# Autodesk Inventor assembly: MotorPulley_Turret
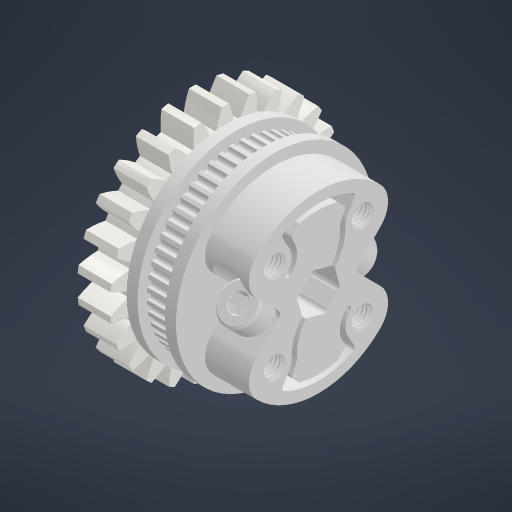
[picture p0: Inventor's stored thumbnail of the model, 512x512]
Saved by Autodesk Inventor 2024 (Build 280153000, 153)
## iProperties
Created: 2023-10-26
Part Number: MotorPulley_Turret
Document SubType Name: Assembly
Designer: avsar
Author: avsar
## Documents named in this file (4)
- C:\Users\avsar\Documents\Inventor\RCR_Arm_Temp\Arm\Turret\MotorPulley_Turret.iam
- C:\Users\avsar\Documents\Inventor\RCR_Arm_Temp\Arm\Turret\MotorConnectionPulley.ipt
- C:\Users\avsar\Documents\Inventor\RCR_Arm_Temp\Arm\Turret\TurretGear.ipt
- C:\Users\avsar\Documents\Inventor\RCR_Arm_Temp\COTS\goBilda\Motion\Hubs\Sonic Hubs\Sonic Hub (8mm REX Bore).ipt
## Components (3 placed, 3 different names)
1. MotorConnectionPulley:1 — Mate:1, Mate:2, Mate:3, Mate:4, Mate:5, Mate:6
2. Sonic Hub (8mm REX Bore):1 — Mate:4, Mate:5, Mate:6
3. Spur Gear1:1 — Mate:1, Mate:2, Mate:3
## Relationships (6: Mate 6)
- Mate:1: MotorConnectionPulley:1 ↔ Spur Gear1:1
- Mate:2: MotorConnectionPulley:1 ↔ Spur Gear1:1
- Mate:3: MotorConnectionPulley:1 ↔ Spur Gear1:1
- Mate:4: MotorConnectionPulley:1 ↔ Sonic Hub (8mm REX Bore):1
- Mate:5: MotorConnectionPulley:1 ↔ Sonic Hub (8mm REX Bore):1
- Mate:6: MotorConnectionPulley:1 ↔ Sonic Hub (8mm REX Bore):1
